# Autodesk Inventor assembly: Assembly1
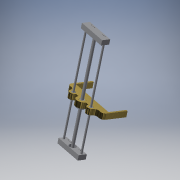
[picture p0: Inventor's stored thumbnail of the model, 180x180]
Saved by Autodesk Inventor 2018 (Build 220112000, 112)
## iProperties
Created: 2017-10-12
Part Number: Assembly1
Document SubType Name: Assembly
Designer: 1452927
Author: 1452927
## Documents named in this file (10)
- D:\FTC\2019-2020\7729-CAD\robot\old_lift\lift_assm.iam
- D:\FTC\2019-2020\7729-CAD\robot\old_lift\SpinnyPiece.ipt
- D:\FTC\2019-2020\7729-CAD\robot\old_lift\SpiralRod.ipt
- D:\FTC\2019-2020\7729-CAD\robot\old_lift\Rod.ipt
- D:\FTC\2019-2020\7729-CAD\robot\old_lift\BearingThing.ipt
- D:\FTC\2019-2020\7729-CAD\robot\old_lift\RodBase.ipt
- D:\FTC\2019-2020\7729-CAD\robot\old_lift\AlteredPlatform.ipt
- D:\FTC\2019-2020\7729-CAD\robot\old_lift\BoxHolders.ipt
- H:\Robotics\lift\BlockCase.ipt
- H:\Robotics\FoamBlock.ipt
## Components (14 placed, 9 different names)
1. SpiralRod:1 — Insert:14, Mate:19, Insert:22, Insert:24, Insert:26
2. Rod:1 — Insert:23, Insert:27
3. Rod:2 — Mate:12, Insert:15, Insert:25, Insert:28
4. BearingThing:1 — Mate:20, Insert:18
5. BearingThing:2 — Mate:12, Insert:19
6. SpinnyPiece:1 — Mate:19, Insert:17
7. RodBase:1 — Insert:14, Insert:15, Insert:23, Insert:24, Insert:25
8. AlteredPlatform:1 — Insert:17, Mate:20, Insert:18, Insert:19, Flush:1, Flush:2, Mate:22, Flush:6, Mate:23
9. RodBase:2 — Insert:22, Insert:26, Insert:27, Insert:28
10. BoxHolders:1 — Flush:1, Flush:2, Mate:22, Flush:7
11. BlockCase:1
12. FoamBlock:1
13. FoamBlock:2
14. BoxHolders:2 — Flush:6, Flush:7, Mate:23
## Relationships (21: Insert 12, Mate 5, Flush 4)
- Mate:12: Rod:2 ↔ BearingThing:2
- Insert:14: SpiralRod:1 ↔ RodBase:1
- Insert:15: Rod:2 ↔ RodBase:1
- Mate:19: SpiralRod:1 ↔ SpinnyPiece:1
- Insert:17: SpinnyPiece:1 ↔ AlteredPlatform:1
- Mate:20: BearingThing:1 ↔ AlteredPlatform:1
- Insert:18: BearingThing:1 ↔ AlteredPlatform:1
- Insert:19: BearingThing:2 ↔ AlteredPlatform:1
- Insert:22: SpiralRod:1 ↔ RodBase:2
- Flush:1: AlteredPlatform:1 ↔ BoxHolders:1
- Flush:2: AlteredPlatform:1 ↔ BoxHolders:1
- Mate:22 (101.6 mm): AlteredPlatform:1 ↔ BoxHolders:1
- Flush:6: AlteredPlatform:1 ↔ BoxHolders:2
- Flush:7: BoxHolders:1 ↔ BoxHolders:2
- Mate:23 (101.6 mm): AlteredPlatform:1 ↔ BoxHolders:2
- Insert:23: Rod:1 ↔ RodBase:1
- Insert:24: SpiralRod:1 ↔ RodBase:1
- Insert:25: Rod:2 ↔ RodBase:1
- Insert:26: SpiralRod:1 ↔ RodBase:2
- Insert:27: Rod:1 ↔ RodBase:2
- Insert:28: Rod:2 ↔ RodBase:2
